# Autodesk Inventor assembly: Sestava
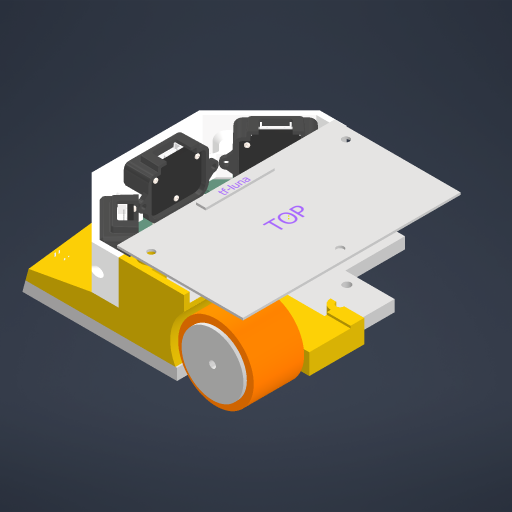
[picture p0: Inventor's stored thumbnail of the model, 512x512]
Saved by Autodesk Inventor 2024 (Build 280153000, 153)
## iProperties
Created: 2024-01-31
Part Number: Sestava
Document SubType Name: Assembly
Designer: Simak
Author: Simak
## Documents named in this file (8)
- C:\Users\Simak\OneDrive\Dokumenty\GitHub\RoboCop\- 3D -\_wip\Sestava.iam
- C:\Users\Simak\OneDrive\Dokumenty\GitHub\RoboCop\- 3D -\mech._parts\base_plate_v2.ipt
- C:\Users\Simak\OneDrive\Dokumenty\GitHub\RoboCop\- 3D -\archive\TF-Luna_holder_v1\Sestava TF-Luna a držáku.iam
- C:\Users\Simak\OneDrive\Dokumenty\GitHub\RoboCop\- 3D -\PCBs\QRE MiniBoards\QRE MiniBoards\QRE_MiniBoards_Board.iam
- C:\Users\Simak\OneDrive\Dokumenty\GitHub\RoboCop\- 3D -\_wip\body.ipt
- C:\Users\Simak\OneDrive\Dokumenty\GitHub\RoboCop\- 3D -\mech._parts\box.ipt
- C:\Users\Simak\OneDrive\Dokumenty\GitHub\RoboCop\- 3D -\mech._parts\JSUMO_Wheel_33x25mm.ipt
- C:\Users\Simak\OneDrive\Dokumenty\GitHub\RoboCop\- 3D -\_wip\pcb_layout\pcb.ipt
## Components (8 placed, 7 different names)
1. base_plate_v2:1 — Proti sobě:2, Stejný směr:1, Proti sobě:3, Stejný směr:2, Vložit:1, Proti sobě:4, Stejný směr:3, Stejný směr:4, Proti sobě:7, Proti sobě:8, Proti sobě:9
2. Sestava TF-Luna a držáku:1 [sub-assembly] — Proti sobě:2, Stejný směr:1, Proti sobě:5, Proti sobě:6, Proti sobě:13
3. QRE_MiniBoards_Board:1 [sub-assembly] — Proti sobě:3, Stejný směr:2, Vložit:1
4. body:1 — Proti sobě:4, Stejný směr:3, Stejný směr:4, Proti sobě:5, Proti sobě:6, Stejný směr:5, Proti sobě:12, Stejný směr:6
5. box:1 — Proti sobě:7, Proti sobě:8, Proti sobě:9, Proti sobě:10, Tečnost:1, Tečnost:2
6. JSUMO_Wheel_33x25mm:1 — Stejný směr:5, Proti sobě:11
7. JSUMO_Wheel_33x25mm:2 — Proti sobě:10, Tečnost:1, Tečnost:2, Proti sobě:11
8. pcb:1 — Proti sobě:12, Stejný směr:6, Proti sobě:13
## Relationships (21: Mate 12, Flush 6, Tangent 2, Insert 1)
- Proti sobě:2 [Mate]: base_plate_v2:1 ↔ Sestava TF-Luna a držáku:1
- Stejný směr:1 [Flush]: base_plate_v2:1 ↔ Sestava TF-Luna a držáku:1
- Proti sobě:3 [Mate] (1 mm): base_plate_v2:1 ↔ QRE_MiniBoards_Board:1
- Stejný směr:2 [Flush] (4.75 mm): base_plate_v2:1 ↔ QRE_MiniBoards_Board:1
- Vložit:1 [Insert]: base_plate_v2:1 ↔ QRE_MiniBoards_Board:1
- Proti sobě:4 [Mate]: base_plate_v2:1 ↔ body:1
- Stejný směr:3 [Flush]: base_plate_v2:1 ↔ body:1
- Stejný směr:4 [Flush]: base_plate_v2:1 ↔ body:1
- Proti sobě:5 [Mate]: Sestava TF-Luna a držáku:1 ↔ body:1
- Proti sobě:6 [Mate]: Sestava TF-Luna a držáku:1 ↔ body:1
- Proti sobě:7 [Mate] (2.5 mm): base_plate_v2:1 ↔ box:1
- Proti sobě:8 [Mate]: base_plate_v2:1 ↔ box:1
- Proti sobě:9 [Mate]: base_plate_v2:1 ↔ box:1
- Proti sobě:10 [Mate]: box:1 ↔ JSUMO_Wheel_33x25mm:2
- Tečnost:1 [Tangent]: box:1 ↔ JSUMO_Wheel_33x25mm:2
- Tečnost:2 [Tangent]: box:1 ↔ JSUMO_Wheel_33x25mm:2
- Stejný směr:5 [Flush]: body:1 ↔ JSUMO_Wheel_33x25mm:1
- Proti sobě:11 [Mate]: JSUMO_Wheel_33x25mm:1 ↔ JSUMO_Wheel_33x25mm:2
- Proti sobě:12 [Mate] (1 mm): body:1 ↔ pcb:1
- Stejný směr:6 [Flush] (2.25 mm): body:1 ↔ pcb:1
- Proti sobě:13 [Mate] (-3 mm): Sestava TF-Luna a držáku:1 ↔ pcb:1
## Named parameters: Finish1_Area = 2.15
note: some values were not read from the file. Shown as the stored number, unit unknown: "Finish1_Area".
